# Autodesk Inventor assembly: Footassembly
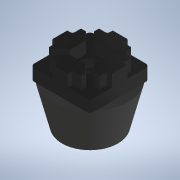
[picture p0: Inventor's stored thumbnail of the model, 180x180]
Saved by Autodesk Inventor 2020.2 (Build 242310000, 310)
## iProperties
Created: 2020-08-24
Part Number: Footassembly
Document SubType Name: Assembly
Designer: JK
Author: JK
## Documents named in this file (3)
- C:\Users\JK\Documents\Inventor\Anet Upgrade\Footassembly.iam
- C:\Users\JK\Documents\Inventor\Anet Upgrade\endcapfoot.ipt
- C:\Users\JK\Documents\Inventor\Anet Upgrade\Rubberfoot.ipt
## Components (2 placed, 2 different names)
1. endcapfoot:1 — Mate:1, Mate:2
2. Rubberfoot:1 — Mate:1, Mate:2
## Relationships (2: Mate 2)
- Mate:1: endcapfoot:1 ↔ Rubberfoot:1
- Mate:2: endcapfoot:1 ↔ Rubberfoot:1
